# Autodesk Inventor assembly: CIM Motor Bane Bot 1764
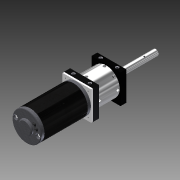
[picture p0: Inventor's stored thumbnail of the model, 180x180]
Saved by Autodesk Inventor 2011 (Build 150239000, 239)
## iProperties
Created: 2008-01-16
Part Number: CIM Motor Bane Bot 1764
Document SubType Name: Assembly
Designer: clee1
Author: clee1
## Documents named in this file (8)
- R:\CAD Archives\Motors\CIM Motor Bane Bots 1764\CIM Motor Bane Bot 1764.iam
- R:\CAD Archives\Motors\CIM Motor Bane Bots 1764\BB2-InterfacePlate 1764.ipt
- R:\CAD Archives\Motors\CIM Motor Bane Bots 1764\BB2-BackPlate 1764.ipt
- R:\CAD Archives\Motors\CIM Motor Bane Bots 1764\BB2-FrontPlate 1764.ipt
- R:\CAD Archives\Motors\CIM Motor Bane Bots 1764\CIM Bearing 1764.ipt
- R:\CAD Archives\Motors\CIM Motor Bane Bots 1764\BB2-RingGear 1764.ipt
- R:\CAD Archives\Motors\CIM Motor Bane Bots 1764\BB2-OutputShaft 2008 Cut 1764.ipt
- R:\CAD Archives\Motors\CIM Motor Bane Bots 1764\CIM Motor 1764.ipt
## Components (8 placed, 7 different names)
1. BB2-InterfacePlate 1764:1 — Mate:1, Flush:1, Flush:2, Mate:12
2. BB2-BackPlate 1764:1 — Mate:1, Flush:1, Flush:2, Mate:5, Mate:6, Angle:1, Angle:2, Mate:11, Angle:4, Flush:3, Flush:4
3. BB2-FrontPlate 1764:1 — Angle:2, Tangent:1, Tangent:2, Mate:13, Flush:3, Flush:4, Flush:5
4. CIM Bearing 1764:3 — Mate:3, Tangent:2
5. CIM Bearing 1764:4 — Mate:3, Tangent:1, Tangent:3, Flush:5, Mate:14
6. BB2-RingGear 1764:1 — Mate:5, Mate:6, Angle:1, Mate:13
7. BB2-OutputShaft 2008 Cut 1764:1 — Tangent:3, Mate:14, Mate:15
8. CIM Motor 1764:1 — Mate:11, Angle:4, Mate:12, Mate:15
## Relationships (20: Mate 9, Flush 5, Angle 3, Tangent 3)
- Mate:1: BB2-InterfacePlate 1764:1 ↔ BB2-BackPlate 1764:1
- Flush:1: BB2-InterfacePlate 1764:1 ↔ BB2-BackPlate 1764:1
- Flush:2: BB2-InterfacePlate 1764:1 ↔ BB2-BackPlate 1764:1
- Mate:3: CIM Bearing 1764:3 ↔ CIM Bearing 1764:4
- Mate:5: BB2-BackPlate 1764:1 ↔ BB2-RingGear 1764:1
- Mate:6: BB2-BackPlate 1764:1 ↔ BB2-RingGear 1764:1
- Angle:1 (0 deg): BB2-BackPlate 1764:1 ↔ BB2-RingGear 1764:1
- Angle:2 (0 deg): BB2-BackPlate 1764:1 ↔ BB2-FrontPlate 1764:1
- Mate:11: BB2-BackPlate 1764:1 ↔ CIM Motor 1764:1
- Angle:4 (0 deg): BB2-BackPlate 1764:1 ↔ CIM Motor 1764:1
- Mate:12: BB2-InterfacePlate 1764:1 ↔ CIM Motor 1764:1
- Tangent:1: BB2-FrontPlate 1764:1 ↔ CIM Bearing 1764:4
- Tangent:2: BB2-FrontPlate 1764:1 ↔ CIM Bearing 1764:3
- Mate:13: BB2-FrontPlate 1764:1 ↔ BB2-RingGear 1764:1
- Flush:3: BB2-BackPlate 1764:1 ↔ BB2-FrontPlate 1764:1
- Tangent:3: CIM Bearing 1764:4 ↔ BB2-OutputShaft 2008 Cut 1764:1
- Flush:4: BB2-BackPlate 1764:1 ↔ BB2-FrontPlate 1764:1
- Flush:5: BB2-FrontPlate 1764:1 ↔ CIM Bearing 1764:4
- Mate:14: CIM Bearing 1764:4 ↔ BB2-OutputShaft 2008 Cut 1764:1
- Mate:15 (7.3152 mm): BB2-OutputShaft 2008 Cut 1764:1 ↔ CIM Motor 1764:1
